# Autodesk Inventor assembly: convayer ammebily
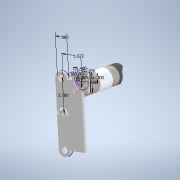
[picture p0: Inventor's stored thumbnail of the model, 180x180]
Saved by Autodesk Inventor 2021 (Build 250183000, 183)
## iProperties
Created: 2021-01-23
Part Number: convayer ammebily
Document SubType Name: Assembly
Designer: User
Author: User
## Documents named in this file (3)
- C:\Robotics\CAD\2020-21-CAD\intake\convayer ammebily.iam
- C:\Robotics\CAD\2020-21-CAD\custom parts\new conveyor bar.ipt
- C:\Robotics\CAD\COTSParts\Motors\am-3102NeveRest20 (1).ipt
## Components (2 placed, 2 different names)
1. new conveyor bar:1 — Mate:1, Mate:2, Mate:3
2. am-3102NeveRest20 (1):1 — Mate:1, Mate:2, Mate:3
## Relationships (3: Mate 3)
- Mate:1: new conveyor bar:1 ↔ am-3102NeveRest20 (1):1
- Mate:2: new conveyor bar:1 ↔ am-3102NeveRest20 (1):1
- Mate:3: new conveyor bar:1 ↔ am-3102NeveRest20 (1):1
